# Autodesk Inventor assembly: cabinet
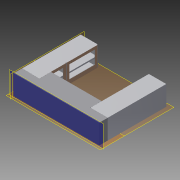
[picture p0: Inventor's stored thumbnail of the model, 180x180]
Saved by Autodesk Inventor 2015 (Build 190159000, 159)
## iProperties
Created: 2015-10-18
Part Number: cabinet
Document SubType Name: Assembly
Designer: omae
Author: omae
## Documents named in this file (3)
- C:\Users\omae\Desktop\研究室\論文・資料\ROS\kitchen\stl\cabinet.iam
- C:\Users\omae\Desktop\研究室\論文・資料\ROS\kitchen\stl\cabinet.ipt
- C:\Users\omae\Desktop\研究室\論文・資料\ROS\kitchen\toolinstall\homeIsland\インポートされたコンポーネント\kitchen cabinet\26.ipt
## Components (3 placed, 2 different names)
1. cabinet:1 — メイト:1, メイト:2, メイト:3, フラッシュ:2, フラッシュ:3, フラッシュ:4, フラッシュ:6
2. 26:1 — フラッシュ:2, フラッシュ:5, フラッシュ:6
3. 26:2 — フラッシュ:3, フラッシュ:4, フラッシュ:5
## Relationships (8: Flush 5, Mate 3)
- メイト:1 [Mate]: cabinet:1
- メイト:2 [Mate]: cabinet:1
- メイト:3 [Mate]: cabinet:1
- フラッシュ:2 [Flush]: cabinet:1 ↔ 26:1
- フラッシュ:3 [Flush]: cabinet:1 ↔ 26:2
- フラッシュ:4 [Flush]: cabinet:1 ↔ 26:2
- フラッシュ:5 [Flush]: 26:1 ↔ 26:2
- フラッシュ:6 [Flush]: cabinet:1 ↔ 26:1
